# Autodesk Inventor assembly: Robot
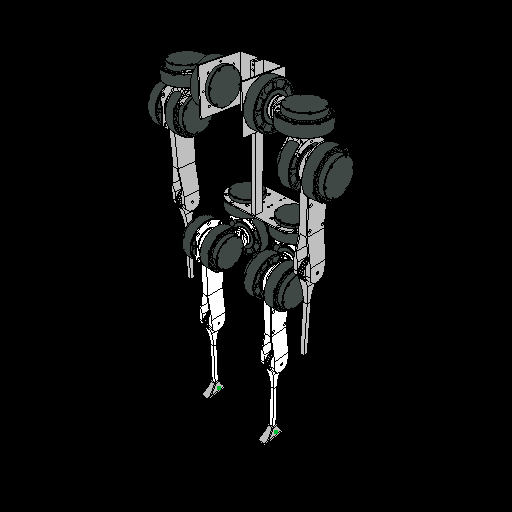
[picture p0: Inventor's stored thumbnail of the model, 512x512]
Saved by Autodesk Inventor 2026 (Build 300175000, 175)
## iProperties
Created: 2025-07-13
Part Number: Robot
Document SubType Name: Assembly
Designer: User
Author: User
## Documents named in this file (28)
- D:\3d parts\robot_v1\Robot.iam
- D:\3d parts\robot_v1\HT-03-Motor.ipt
- D:\3d parts\robot_v1\waist_hip_connector_v3.ipt
- D:\3d parts\robot_v1\waist_hip_joint_v2.ipt
- D:\3d parts\robot_v1\upperleg.ipt
- D:\3d parts\robot_v1\upperleg_gear_side.ipt
- D:\3d parts\robot_v1\18teeth_gear.ipt
- D:\3d parts\robot_v1\18teeth_gear_connector.ipt
- D:\3d parts\robot_v1\Robot\Design Accelerator\Bearing5.iam
- D:\3d parts\robot_v1\28teeth_gear.ipt
- D:\3d parts\robot_v1\lower_leg.ipt
- D:\3d parts\robot_v1\ab_hip_joint_connector.ipt
- D:\3d parts\robot_v1\ab_hip_connector.ipt
- D:\3d parts\robot_v1\HT-03-Motor_MIR.ipt
- D:\3d parts\robot_v1\waist_hip_joint_v2_MIR.ipt
- D:\3d parts\robot_v1\waist_hip_connector_v3_MIR.ipt
- D:\3d parts\robot_v1\upperleg_MIR.ipt
- D:\3d parts\robot_v1\upperleg_gear_side_MIR.ipt
- D:\3d parts\robot_v1\18teeth_gear_connector_MIR.ipt
- D:\3d parts\robot_v1\18teeth_gear_MIR.ipt
- D:\3d parts\robot_v1\28teeth_gear_MIR.ipt
- D:\3d parts\robot_v1\lower_leg_MIR.ipt
- D:\3d parts\robot_v1\ab_hip_joint_connector_MIR.ipt
- D:\3d parts\robot_v1\ab_hip_connector_MIR.ipt
- D:\3d parts\robot_v1\leg_connector.ipt
- D:\3d parts\robot_v1\foot.ipt
- D:\3d parts\robot_v1\shoulder.ipt
- D:\3d parts\robot_v1\spine.ipt
## Components (65 placed, 27 different names)
1. HT-03-Motor:1 — Rotational:1, Mate:29, Mate:30, Mate:31
2. HT-03-Motor:2 — Mate:4, Mate:5, Mate:6, Rotational:2
3. waist_hip_joint_v2:1 — Mate:1, Mate:2, Mate:3, Rotational:1
4. waist_hip_connector_v3:1 — Mate:1, Mate:2, Mate:3, Mate:4, Mate:5, Mate:6
5. upperleg:1 — Rotational:2, Mate:10, Mate:11, Mate:12, Rotational:4
6. HT-03-Motor:3 — Mate:13, Mate:14, Mate:15, Rotational:3
7. upperleg_gear_side:1 — Mate:10, Mate:11, Mate:12, Mate:13, Mate:14, Mate:15
8. 18teeth_gear_connector:1 — Mate:16, Mate:17, Rotational:3, Mate:23
9. 18teeth_gear:1 — Mate:16, Mate:17, Mate:23
10. Bearing:1 [sub-assembly] — Mate:19, Mate:20, Rotational:4
11. 28teeth_gear:1 — Mate:19, Mate:20, Mate:21, Mate:22, Mate:24, Mate:25
12. Bearing:2 [sub-assembly] — Mate:21, Mate:22
13. lower_leg:1 — Mate:24, Mate:25, Mate:65, Mate:66, Mate:67
14. HT-03-Motor:4 — Rotational:5, Mate:59, Mate:60, Mate:61
15. ab_hip_joint_connector:1 — Mate:26, Mate:27, Mate:28, Rotational:5
16. ab_hip_connector:1 — Mate:26, Mate:27, Mate:28, Mate:29, Mate:30, Mate:31
17. HT-03-Motor_MIR:1 — Mate:53, Mate:54, Mate:55, Rotational:6
18. HT-03-Motor_MIR:2 — Mate:32, Mate:33, Mate:34, Rotational:7
19. waist_hip_joint_v2_MIR:1 — Mate:35, Mate:36, Mate:37, Rotational:6
20. waist_hip_connector_v3_MIR:1 — Mate:32, Mate:33, Mate:34, Mate:35, Mate:36, Mate:37
21. upperleg_MIR:1 — Mate:38, Mate:42, Mate:43, Rotational:7, Rotational:9
22. HT-03-Motor_MIR:3 — Mate:39, Mate:40, Mate:41, Rotational:8
23. upperleg_gear_side_MIR:1 — Mate:38, Mate:39, Mate:40, Mate:41, Mate:42, Mate:43
24. 18teeth_gear_connector_MIR:1 — Mate:44, Mate:45, Mate:46, Rotational:8
25. 18teeth_gear_MIR:1 — Mate:44, Mate:45, Mate:46
26. Bearing:3 [sub-assembly] — Mate:47, Mate:48, Rotational:9
27. 28teeth_gear_MIR:1 — Mate:47, Mate:48, Mate:49, Mate:50, Mate:51, Mate:52
28. Bearing:4 [sub-assembly] — Mate:49, Mate:50
29. lower_leg_MIR:1 — Mate:51, Mate:52, Mate:68, Mate:69, Mate:70
30. HT-03-Motor_MIR:4 — Rotational:10, Mate:62, Mate:63, Mate:64
31. ab_hip_joint_connector_MIR:1 — Mate:56, Mate:57, Mate:58, Rotational:10
32. ab_hip_connector_MIR:1 — Mate:53, Mate:54, Mate:55, Mate:56, Mate:57, Mate:58
33. leg_connector:1 — Mate:59, Mate:60, Mate:61, Mate:62, Mate:63, Mate:64, Mate:92, Mate:119, Mate:120
34. foot:1 — Mate:65, Mate:66, Mate:67
35. foot:2 — Mate:68, Mate:69, Mate:70
36. shoulder:1 — Mate:89, Mate:90, Mate:91, Mate:95, Mate:96, Mate:97, Mate:116, Mate:117, Mate:118
37. HT-03-Motor:5
38. HT-03-Motor:6
39. waist_hip_joint_v2:2
40. waist_hip_connector_v3:2
41. upperleg:2 — Rotational:17
42. HT-03-Motor:7
43. upperleg_gear_side:2
44. HT-03-Motor:8 — Mate:89, Mate:90, Mate:91
45. ab_hip_joint_connector:2
46. ab_hip_connector:2
47. spine:1 — Mate:92, Mate:95, Mate:96, Mate:97, Mate:119, Mate:120
48. HT-03-Motor_MIR:5
49. HT-03-Motor_MIR:6
50. waist_hip_joint_v2_MIR:2
51. waist_hip_connector_v3_MIR:2
52. upperleg_MIR:2 — Rotational:18
53. HT-03-Motor_MIR:7
54. upperleg_gear_side_MIR:2
55. HT-03-Motor_MIR:8 — Mate:116, Mate:117, Mate:118
56. ab_hip_joint_connector_MIR:2
57. ab_hip_connector_MIR:2
58. Bearing:5 [sub-assembly]
59. 28teeth_gear:2 — Rotational:17
60. Bearing:6 [sub-assembly]
61. lower_leg:2
62. Bearing:7 [sub-assembly]
63. 28teeth_gear:3
64. Bearing:8 [sub-assembly] — Rotational:18
65. lower_leg:3
## Relationships (144: Mate 126, RevoluteJoint 18)
- Mate:1: waist_hip_joint_v2:1 ↔ waist_hip_connector_v3:1
- Mate:2: waist_hip_joint_v2:1 ↔ waist_hip_connector_v3:1
- Mate:3: waist_hip_joint_v2:1 ↔ waist_hip_connector_v3:1
- Rotational:1 [RevoluteJoint]: HT-03-Motor:1 ↔ waist_hip_joint_v2:1
- Mate:4: HT-03-Motor:2 ↔ waist_hip_connector_v3:1
- Mate:5: HT-03-Motor:2 ↔ waist_hip_connector_v3:1
- Mate:6: HT-03-Motor:2 ↔ waist_hip_connector_v3:1
- Rotational:2 [RevoluteJoint]: HT-03-Motor:2 ↔ upperleg:1
- Mate:10: upperleg:1 ↔ upperleg_gear_side:1
- Mate:11: upperleg:1 ↔ upperleg_gear_side:1
- Mate:12: upperleg:1 ↔ upperleg_gear_side:1
- Mate:13: HT-03-Motor:3 ↔ upperleg_gear_side:1
- Mate:14: HT-03-Motor:3 ↔ upperleg_gear_side:1
- Mate:15: HT-03-Motor:3 ↔ upperleg_gear_side:1
- Mate:16: 18teeth_gear_connector:1 ↔ 18teeth_gear:1
- Mate:17: 18teeth_gear_connector:1 ↔ 18teeth_gear:1
- Rotational:3 [RevoluteJoint]: HT-03-Motor:3 ↔ 18teeth_gear_connector:1
- Mate:19: Bearing:1 ↔ 28teeth_gear:1
- Mate:20: Bearing:1 ↔ 28teeth_gear:1
- Mate:21: 28teeth_gear:1 ↔ Bearing:2
- Mate:22: 28teeth_gear:1 ↔ Bearing:2
- Mate:23: 18teeth_gear_connector:1 ↔ 18teeth_gear:1
- Rotational:4 [RevoluteJoint]: upperleg:1 ↔ Bearing:1
- Mate:24: 28teeth_gear:1 ↔ lower_leg:1
- Mate:25: 28teeth_gear:1 ↔ lower_leg:1
- Mate:26: ab_hip_joint_connector:1 ↔ ab_hip_connector:1
- Mate:27: ab_hip_joint_connector:1 ↔ ab_hip_connector:1
- Mate:28: ab_hip_joint_connector:1 ↔ ab_hip_connector:1
- Rotational:5 [RevoluteJoint]: HT-03-Motor:4 ↔ ab_hip_joint_connector:1
- Mate:29: HT-03-Motor:1 ↔ ab_hip_connector:1
- Mate:30: HT-03-Motor:1 ↔ ab_hip_connector:1
- Mate:31: HT-03-Motor:1 ↔ ab_hip_connector:1
- Mate:32: HT-03-Motor_MIR:2 ↔ waist_hip_connector_v3_MIR:1
- Mate:33: HT-03-Motor_MIR:2 ↔ waist_hip_connector_v3_MIR:1
- Mate:34: HT-03-Motor_MIR:2 ↔ waist_hip_connector_v3_MIR:1
- Mate:35: waist_hip_joint_v2_MIR:1 ↔ waist_hip_connector_v3_MIR:1
- Mate:36: waist_hip_joint_v2_MIR:1 ↔ waist_hip_connector_v3_MIR:1
- Mate:37: waist_hip_joint_v2_MIR:1 ↔ waist_hip_connector_v3_MIR:1
- Mate:38: upperleg_MIR:1 ↔ upperleg_gear_side_MIR:1
- Mate:39: HT-03-Motor_MIR:3 ↔ upperleg_gear_side_MIR:1
- Mate:40: HT-03-Motor_MIR:3 ↔ upperleg_gear_side_MIR:1
- Mate:41: HT-03-Motor_MIR:3 ↔ upperleg_gear_side_MIR:1
- Mate:42: upperleg_MIR:1 ↔ upperleg_gear_side_MIR:1
- Mate:43: upperleg_MIR:1 ↔ upperleg_gear_side_MIR:1
- Mate:44: 18teeth_gear_connector_MIR:1 ↔ 18teeth_gear_MIR:1
- Mate:45: 18teeth_gear_connector_MIR:1 ↔ 18teeth_gear_MIR:1
- Mate:46: 18teeth_gear_connector_MIR:1 ↔ 18teeth_gear_MIR:1
- Mate:47: Bearing:3 ↔ 28teeth_gear_MIR:1
- Mate:48: Bearing:3 ↔ 28teeth_gear_MIR:1
- Mate:49: 28teeth_gear_MIR:1 ↔ Bearing:4
- Mate:50: 28teeth_gear_MIR:1 ↔ Bearing:4
- Mate:51: 28teeth_gear_MIR:1 ↔ lower_leg_MIR:1
- Mate:52: 28teeth_gear_MIR:1 ↔ lower_leg_MIR:1
- Mate:53: HT-03-Motor_MIR:1 ↔ ab_hip_connector_MIR:1
- Mate:54: HT-03-Motor_MIR:1 ↔ ab_hip_connector_MIR:1
- Mate:55: HT-03-Motor_MIR:1 ↔ ab_hip_connector_MIR:1
- Mate:56: ab_hip_joint_connector_MIR:1 ↔ ab_hip_connector_MIR:1
- Mate:57: ab_hip_joint_connector_MIR:1 ↔ ab_hip_connector_MIR:1
- Mate:58: ab_hip_joint_connector_MIR:1 ↔ ab_hip_connector_MIR:1
- Rotational:6 [RevoluteJoint]: HT-03-Motor_MIR:1 ↔ waist_hip_joint_v2_MIR:1
- Rotational:7 [RevoluteJoint]: HT-03-Motor_MIR:2 ↔ upperleg_MIR:1
- Rotational:8 [RevoluteJoint]: HT-03-Motor_MIR:3 ↔ 18teeth_gear_connector_MIR:1
- Rotational:9 [RevoluteJoint]: upperleg_MIR:1 ↔ Bearing:3
- Rotational:10 [RevoluteJoint]: HT-03-Motor_MIR:4 ↔ ab_hip_joint_connector_MIR:1
- Mate:59: HT-03-Motor:4 ↔ leg_connector:1
- Mate:60: HT-03-Motor:4 ↔ leg_connector:1
- Mate:61: HT-03-Motor:4 ↔ leg_connector:1
- Mate:62: HT-03-Motor_MIR:4 ↔ leg_connector:1
- Mate:63: HT-03-Motor_MIR:4 ↔ leg_connector:1
- Mate:64: HT-03-Motor_MIR:4 ↔ leg_connector:1
- Mate:65: lower_leg:1 ↔ foot:1
- Mate:66: lower_leg:1 ↔ foot:1
- Mate:67: lower_leg:1 ↔ foot:1
- Mate:68: lower_leg_MIR:1 ↔ foot:2
- Mate:69: lower_leg_MIR:1 ↔ foot:2
- Mate:70: lower_leg_MIR:1 ↔ foot:2
- [Mate]: waist_hip_joint_v2:2 ↔ waist_hip_connector_v3:2
- [Mate]: waist_hip_joint_v2:2 ↔ waist_hip_connector_v3:2
- [Mate]: waist_hip_joint_v2:2 ↔ waist_hip_connector_v3:2
- [RevoluteJoint]: HT-03-Motor:5 ↔ waist_hip_joint_v2:2
- [Mate]: HT-03-Motor:6 ↔ waist_hip_connector_v3:2
- [Mate]: HT-03-Motor:6 ↔ waist_hip_connector_v3:2
- [Mate]: HT-03-Motor:6 ↔ waist_hip_connector_v3:2
- [RevoluteJoint]: HT-03-Motor:6 ↔ upperleg:2
- [Mate]: upperleg:2 ↔ upperleg_gear_side:2
- [Mate]: upperleg:2 ↔ upperleg_gear_side:2
- [Mate]: upperleg:2 ↔ upperleg_gear_side:2
- [Mate]: HT-03-Motor:7 ↔ upperleg_gear_side:2
- [Mate]: HT-03-Motor:7 ↔ upperleg_gear_side:2
- [Mate]: HT-03-Motor:7 ↔ upperleg_gear_side:2
- [Mate]: ab_hip_joint_connector:2 ↔ ab_hip_connector:2
- [Mate]: ab_hip_joint_connector:2 ↔ ab_hip_connector:2
- [Mate]: ab_hip_joint_connector:2 ↔ ab_hip_connector:2
- [RevoluteJoint]: HT-03-Motor:8 ↔ ab_hip_joint_connector:2
- [Mate]: HT-03-Motor:5 ↔ ab_hip_connector:2
- [Mate]: HT-03-Motor:5 ↔ ab_hip_connector:2
- [Mate]: HT-03-Motor:5 ↔ ab_hip_connector:2
- Mate:89: shoulder:1 ↔ HT-03-Motor:8
- Mate:90: shoulder:1 ↔ HT-03-Motor:8
- Mate:91: shoulder:1 ↔ HT-03-Motor:8
- Mate:92: leg_connector:1 ↔ spine:1
- Mate:95: shoulder:1 ↔ spine:1
- Mate:96: shoulder:1 ↔ spine:1
- Mate:97: shoulder:1 ↔ spine:1
- [Mate]: HT-03-Motor_MIR:6 ↔ waist_hip_connector_v3_MIR:2
- [Mate]: HT-03-Motor_MIR:6 ↔ waist_hip_connector_v3_MIR:2
- [Mate]: HT-03-Motor_MIR:6 ↔ waist_hip_connector_v3_MIR:2
- [Mate]: waist_hip_joint_v2_MIR:2 ↔ waist_hip_connector_v3_MIR:2
- [Mate]: waist_hip_joint_v2_MIR:2 ↔ waist_hip_connector_v3_MIR:2
- [Mate]: waist_hip_joint_v2_MIR:2 ↔ waist_hip_connector_v3_MIR:2
- [Mate]: upperleg_MIR:2 ↔ upperleg_gear_side_MIR:2
- [Mate]: HT-03-Motor_MIR:7 ↔ upperleg_gear_side_MIR:2
- [Mate]: HT-03-Motor_MIR:7 ↔ upperleg_gear_side_MIR:2
- [Mate]: HT-03-Motor_MIR:7 ↔ upperleg_gear_side_MIR:2
- [Mate]: upperleg_MIR:2 ↔ upperleg_gear_side_MIR:2
- [Mate]: upperleg_MIR:2 ↔ upperleg_gear_side_MIR:2
- [Mate]: HT-03-Motor_MIR:5 ↔ ab_hip_connector_MIR:2
- [Mate]: HT-03-Motor_MIR:5 ↔ ab_hip_connector_MIR:2
- [Mate]: HT-03-Motor_MIR:5 ↔ ab_hip_connector_MIR:2
- [Mate]: ab_hip_joint_connector_MIR:2 ↔ ab_hip_connector_MIR:2
- [Mate]: ab_hip_joint_connector_MIR:2 ↔ ab_hip_connector_MIR:2
- [Mate]: ab_hip_joint_connector_MIR:2 ↔ ab_hip_connector_MIR:2
- [RevoluteJoint]: HT-03-Motor_MIR:5 ↔ waist_hip_joint_v2_MIR:2
- [RevoluteJoint]: HT-03-Motor_MIR:6 ↔ upperleg_MIR:2
- [RevoluteJoint]: HT-03-Motor_MIR:8 ↔ ab_hip_joint_connector_MIR:2
- Mate:116: shoulder:1 ↔ HT-03-Motor_MIR:8
- Mate:117: shoulder:1 ↔ HT-03-Motor_MIR:8
- Mate:118: shoulder:1 ↔ HT-03-Motor_MIR:8
- Mate:119: leg_connector:1 ↔ spine:1
- Mate:120: leg_connector:1 ↔ spine:1
- [Mate]: Bearing:5 ↔ 28teeth_gear:2
- [Mate]: Bearing:5 ↔ 28teeth_gear:2
- [Mate]: 28teeth_gear:2 ↔ Bearing:6
- [Mate]: 28teeth_gear:2 ↔ Bearing:6
- [Mate]: 28teeth_gear:2 ↔ lower_leg:2
- [Mate]: 28teeth_gear:2 ↔ lower_leg:2
- Rotational:17 [RevoluteJoint]: upperleg:2 ↔ 28teeth_gear:2
- [Mate]: Bearing:7 ↔ 28teeth_gear:3
- [Mate]: Bearing:7 ↔ 28teeth_gear:3
- [Mate]: 28teeth_gear:3 ↔ Bearing:8
- [Mate]: 28teeth_gear:3 ↔ Bearing:8
- [Mate]: 28teeth_gear:3 ↔ lower_leg:3
- [Mate]: 28teeth_gear:3 ↔ lower_leg:3
- Rotational:18 [RevoluteJoint]: upperleg_MIR:2 ↔ Bearing:8
## Named parameters: d227_d132 = 0 mm, d228_d134 = 0 mm, d229_d135 = 0 mm, d230_d136 = 0 mm, d231_d137 = -170.949768 deg, d232_d138 = 0 mm, d233_d139 = 0 mm, d234_d140 = 0 mm, d235_d95 = 0 mm, d236_d96 = 0 mm, d237_d97 = 0 mm, d238_d99 = 0 mm, d239_d100 = 0 mm, d240_d102 = 0 mm, d241_d54 = 0 mm, d242_d56 = 0 mm, d243_d57 = 0 mm, d244_d58 = 0 mm, d245_d59 = -115.597226 deg, d246_d60 = 0 mm, d247_d61 = 0 mm, d248_d62 = 0 mm, d249_d63 = 0 mm, d250_d64 = 83.602955 deg, d260_d162 = 0 mm, d261_d163 = 0 mm, d262_d164 = 0 mm, d263_d165 = 0 mm, d264_d166 = 0 mm, d265_d167 = 0 mm, d266_d168 = 0 mm, d267_d169 = 114.244656 deg, d268_d170 = 0 mm, d269_d171 = -84.460839 deg, d270_d176 = 0 mm, d271_d177 = -54.374538 deg, d272_d141 = 0 mm, d273_d142 = 0 mm, d274_d143 = 0 mm, d275_d144 = 0 mm, d276_d145 = 0 mm, d277_d146 = 0 mm, d278_d147 = 0 mm, d279_d148 = 0 mm, d280_d149 = 0 mm, d281_d150 = 0 mm, d282_d151 = 0 mm, d283_d152 = 0 mm, d289_d128 = 0 mm, d290_d129 = 0 mm, d291_d112 = 0 mm, d292_d113 = 0 mm, d293_d114 = 0 mm, d294_d115 = 0 mm, d297_d128 = 0 mm, d298_d129 = 0 mm, d299_d112 = 0 mm, d300_d113 = 0 mm, d301_d114 = 0 mm, d302_d115 = 0 mm
